# Autodesk Inventor assembly: Base_AX12-explosionado
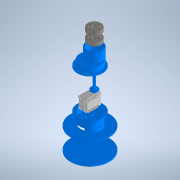
[picture p0: Inventor's stored thumbnail of the model, 180x180]
Saved by Autodesk Inventor 2021 (Build 250183000, 183)
## iProperties
Created: 2022-06-07
Part Number: Base_AX12-explosionado
Document SubType Name: Assembly
Designer: Alcatraz
Author: Alcatraz
## Documents named in this file (7)
- C:\Users\Ivan\Desktop\Nueva carpeta\TESIS\Lista_Piezas_MovPlano_21Junio\Lista_Piezas\Base-AX12\Base_AX12-explosionado.iam
- C:\Users\Ivan\Desktop\Nueva carpeta\TESIS\Lista_Piezas_MovPlano_21Junio\Lista_Piezas\Rodamiento_Giro_V7\Rodamiento_Giro_V7.iam
- C:\Users\Ivan\Desktop\Nueva carpeta\TESIS\Lista_Piezas_MovPlano_21Junio\Lista_Piezas\Base-AX12\B-01.ipt
- C:\Users\Ivan\Desktop\Nueva carpeta\TESIS\Lista_Piezas_MovPlano_21Junio\Lista_Piezas\Base-AX12\B-02.ipt
- C:\Users\Ivan\Desktop\Nueva carpeta\TESIS\Lista_Piezas_MovPlano_21Junio\Lista_Piezas\Base-AX12\B-03.ipt
- C:\Users\Ivan\Desktop\Nueva carpeta\TESIS\Lista_Piezas_MovPlano_21Junio\Lista_Piezas\Bridas\BM-AX12.ipt
- C:\Users\Ivan\Desktop\Nueva carpeta\TESIS\Lista_Piezas_MovPlano_21Junio\Lista_Piezas\AX-12A,18A,12W,MX-12W(stp)\AX-12A.iam
## Components (7 placed, 6 different names)
1. Rodamiento_Giro_V7:1 [sub-assembly] — Coincidencia:4, Coincidencia:12
2. Rodamiento_Giro_V7:2 [sub-assembly] — Coincidencia:4
3. B-01:1 — Coincidencia:14, Coincidencia:15
4. B-02:1 — Coincidencia:1, Coincidencia:2, Coincidencia:6, Coincidencia:7, Coincidencia:14, Coincidencia:15
5. B-03:1 — Coincidencia:6, Coincidencia:7
6. BM-AX12:1 — Coincidencia:9, Coincidencia:10, Coincidencia:11, Coincidencia:12
7. AX-12A:1 [sub-assembly] — Coincidencia:1, Coincidencia:2, Coincidencia:9, Coincidencia:10, Coincidencia:11
## Relationships (11: Mate 11)
- Coincidencia:1 [Mate]: B-02:1 ↔ AX-12A:1
- Coincidencia:2 [Mate]: B-02:1 ↔ AX-12A:1
- Coincidencia:4 [Mate]: Rodamiento_Giro_V7:1 ↔ Rodamiento_Giro_V7:2
- Coincidencia:6 [Mate]: B-02:1 ↔ B-03:1
- Coincidencia:7 [Mate]: B-02:1 ↔ B-03:1
- Coincidencia:9 [Mate]: BM-AX12:1 ↔ AX-12A:1
- Coincidencia:10 [Mate]: BM-AX12:1 ↔ AX-12A:1
- Coincidencia:11 [Mate]: BM-AX12:1 ↔ AX-12A:1
- Coincidencia:12 [Mate]: Rodamiento_Giro_V7:1 ↔ BM-AX12:1
- Coincidencia:14 [Mate]: B-01:1 ↔ B-02:1
- Coincidencia:15 [Mate]: B-01:1 ↔ B-02:1
